# Autodesk Inventor assembly: SpinCoaterAssembly
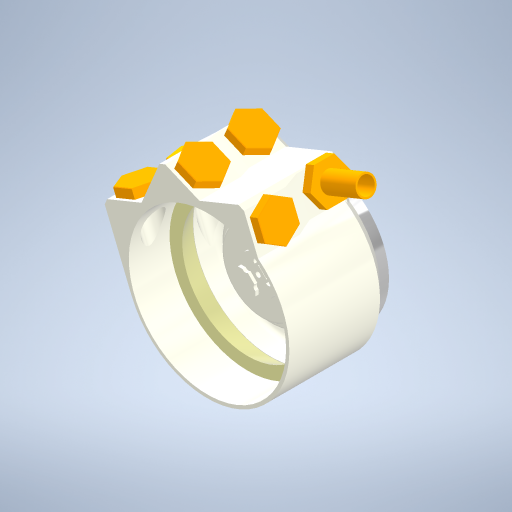
[picture p0: Inventor's stored thumbnail of the model, 512x512]
Saved by Autodesk Inventor 2023.1 (Build 271208000, 208)
## iProperties
Created: 2022-12-04
Part Number: SpinCoaterAssembly
Document SubType Name: Assembly
Designer: Timo
Author: Timo
## Documents named in this file (14)
- C:\Users\Timo\Documents\Inventor\Models\Setups\InSitu\Motor\GloveboxLike\V03\SpinCoaterAssembly\SpinCoaterAssembly.iam
- C:\Users\Timo\Documents\Inventor\Models\Setups\InSitu\Motor\GloveboxLike\V03\SpinCoaterAssembly\Base_Bowl_Glovebox.ipt
- C:\Users\Timo\Documents\Inventor\Models\Setups\InSitu\Motor\GloveboxLike\V03\SpinCoaterAssembly\Bowl_GloveboxLike-small_ScrewingAbove.ipt
- C:\Users\Timo\Documents\Inventor\Models\Setups\InSitu\Motor\GloveboxLike\V03\SpinCoaterAssembly\chuck_v03.ipt
- C:\Users\Timo\Documents\Inventor\Models\Setups\InSitu\Motor\GloveboxLike\V03\SpinCoaterAssembly\Cover.ipt
- C:\Users\Timo\Documents\Inventor\Models\Setups\InSitu\Motor\GloveboxLike\V03\SpinCoaterAssembly\Cover_EqualPressure.ipt
- C:\Users\Timo\Documents\Inventor\Models\Setups\InSitu\Motor\GloveboxLike\V03\SpinCoaterAssembly\Deckel.ipt
- C:\Users\Timo\Documents\Inventor\Models\Setups\InSitu\Motor\GloveboxLike\V03\SpinCoaterAssembly\M24_2_1_4inch.ipt
- C:\Users\Timo\Documents\Inventor\Models\Setups\InSitu\Motor\GloveboxLike\V03\SpinCoaterAssembly\motor.ipt
- C:\Users\Timo\Documents\Inventor\Models\Setups\InSitu\Motor\GloveboxLike\V03\SpinCoaterAssembly\motor_top.ipt
- C:\Users\Timo\Documents\Inventor\Models\Setups\InSitu\Motor\GloveboxLike\V03\SpinCoaterAssembly\MotorHolder.ipt
- C:\Users\Timo\Documents\Inventor\Models\Setups\InSitu\Motor\GloveboxLike\V03\SpinCoaterAssembly\WaterAdapter.ipt
- C:\Users\Timo\Documents\Inventor\Models\Setups\InSitu\Motor\GloveboxLike\V03\SpinCoaterAssembly\WaterAdapter_Closure.ipt
- C:\Users\Timo\Documents\Inventor\Models\Setups\InSitu\Motor\GloveboxLike\V03\SpinCoaterAssembly\Ring.ipt
## Components (16 placed, 13 different names)
1. Base_Bowl_Glovebox:1 — Rigid:2, Rotational:5
2. Bowl_GloveboxLike-small_ScrewingAbove:1 — Rigid:3, Rotational:5, Rigid:6, Rotational:6, Rotational:7, Rotational:8, Rotational:9, Rotational:10, Rotational:11
3. chuck_v03:1 — Rotational:3
4. Cover:1 — Rigid:4, Rigid:5
5. Cover_EqualPressure:1 — Rigid:5
6. Deckel:1 — Rigid:3, Rigid:4
7. M24_2_1_4inch:1 — Rigid:6
8. motor:1 — Rotational:2, Rotational:4
9. motor_top:1 — Rotational:2, Rotational:3
10. MotorHolder:1 — Rigid:2, Rotational:4
11. WaterAdapter:1 — Rotational:6
12. WaterAdapter_Closure:1 — Rotational:7
13. WaterAdapter_Closure:2 — Rotational:8
14. WaterAdapter_Closure:3 — Rotational:9
15. WaterAdapter_Closure:4 — Rotational:10
16. Ring:1 — Rotational:11
## Relationships (15: RevoluteJoint 10, WeldJoint 5)
- Rigid:3 [WeldJoint]: Bowl_GloveboxLike-small_ScrewingAbove:1 ↔ Deckel:1
- Rotational:2 [RevoluteJoint]: motor:1 ↔ motor_top:1
- Rotational:3 [RevoluteJoint]: chuck_v03:1 ↔ motor_top:1
- Rigid:2 [WeldJoint]: Base_Bowl_Glovebox:1 ↔ MotorHolder:1
- Rotational:4 [RevoluteJoint]: motor:1 ↔ MotorHolder:1
- Rotational:5 [RevoluteJoint]: Base_Bowl_Glovebox:1 ↔ Bowl_GloveboxLike-small_ScrewingAbove:1
- Rigid:4 [WeldJoint]: Cover:1 ↔ Deckel:1
- Rigid:5 [WeldJoint]: Cover:1 ↔ Cover_EqualPressure:1
- Rigid:6 [WeldJoint]: Bowl_GloveboxLike-small_ScrewingAbove:1 ↔ M24_2_1_4inch:1
- Rotational:6 [RevoluteJoint]: Bowl_GloveboxLike-small_ScrewingAbove:1 ↔ WaterAdapter:1
- Rotational:7 [RevoluteJoint]: Bowl_GloveboxLike-small_ScrewingAbove:1 ↔ WaterAdapter_Closure:1
- Rotational:8 [RevoluteJoint]: Bowl_GloveboxLike-small_ScrewingAbove:1 ↔ WaterAdapter_Closure:2
- Rotational:9 [RevoluteJoint]: Bowl_GloveboxLike-small_ScrewingAbove:1 ↔ WaterAdapter_Closure:3
- Rotational:10 [RevoluteJoint]: Bowl_GloveboxLike-small_ScrewingAbove:1 ↔ WaterAdapter_Closure:4
- Rotational:11 [RevoluteJoint]: Bowl_GloveboxLike-small_ScrewingAbove:1 ↔ Ring:1
